# Autodesk Inventor assembly: GFRP_T2_08
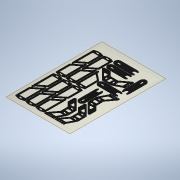
[picture p0: Inventor's stored thumbnail of the model, 180x180]
Saved by Autodesk Inventor 2020 (Build 240168000, 168)
## iProperties
Created: 2021-08-27
Part Number: GFRP_T2_08
Document SubType Name: Assembly
Designer: Masato
Author: Masato
## Documents named in this file (5)
- C:\Users\naoki\Documents\Inventor\CitBrains\git_clone\SUSTAINA_ver1_0\A_T2_175\SUSTAINA-OP\Cam\GFRP_T2_08.iam
- C:\Users\naoki\Documents\Inventor\CitBrains\git_clone\SUSTAINA_ver1_0\A_T2_175\SUSTAINA-OP\Cam\DisposableBoard.ipt
- C:\Users\naoki\Documents\Inventor\CitBrains\git_clone\SUSTAINA_ver1_0\A_T2_175\SUSTAINA-OP\UpperBody\Arm\UpperArm_side_frame.ipt
- C:\Users\naoki\Documents\Inventor\CitBrains\git_clone\SUSTAINA_ver1_0\A_T2_175\SUSTAINA-OP\UpperBody\Head\Head_side_frame.ipt
- C:\Users\naoki\Documents\Inventor\CitBrains\git_clone\SUSTAINA_ver1_0\A_T2_175\SUSTAINA-OP\UpperBody\Arm\ForeArm_inside_frame.ipt
## Components (21 placed, 4 different names)
1. DisposableBoard:1 — メイト:2, メイト:1, フラッシュ:1, フラッシュ:2, フラッシュ:3, メイト:4, メイト:5, フラッシュ:4, メイト:11, メイト:12, メイト:17, フラッシュ:7, メイト:28, メイト:29, メイト:30, フラッシュ:9, メイト:31, メイト:36, メイト:38, メイト:41, メイト:43, メイト:46
2. Head_side_frame:1 — メイト:12, フラッシュ:7, フラッシュ:8, メイト:24, メイト:34, 正接:3
3. Head_side_frame:2 — メイト:11, フラッシュ:8, メイト:24, メイト:26, フラッシュ:11
4. Head_side_frame:3 — メイト:17, メイト:26, メイト:37, フラッシュ:11, メイト:39
5. Head_side_frame:4 — メイト:29, メイト:40, 正接:5, メイト:42, メイト:45
6. UpperArm_side_frame:9 — メイト:30, フラッシュ:9, 正接:2, フラッシュ:10, メイト:34, メイト:35
7. UpperArm_side_frame:10 — 正接:2, メイト:31, フラッシュ:10, メイト:32
8. UpperArm_side_frame:11 — メイト:28, メイト:32, メイト:33, 正接:4
9. ForeArm_inside_frame:1 — メイト:36, 正接:3, メイト:37
10. ForeArm_inside_frame:2 — メイト:38, メイト:39, 正接:4, メイト:40, 正接:8
11. ForeArm_inside_frame:3 — メイト:45, メイト:46, 正接:8
12. ForeArm_inside_frame:4 — メイト:41, メイト:42, 正接:6, メイト:44
13. ForeArm_inside_frame:5 — 正接:7, メイト:43, メイト:44
14. UpperArm_side_frame:1 — メイト:5, フラッシュ:5, 正接:1
15. UpperArm_side_frame:2 — フラッシュ:3, メイト:4, フラッシュ:4, フラッシュ:5, 正接:1
16. UpperArm_side_frame:3
17. UpperArm_side_frame:4
18. UpperArm_side_frame:5
19. UpperArm_side_frame:6 — メイト:35
20. UpperArm_side_frame:7 — 正接:5, 正接:6, 正接:7
21. UpperArm_side_frame:8 — メイト:33
## Component patterns: (4 elements, first: UpperArm_side_frame:1 + UpperArm_side_frame:2)
## Relationships (46: Mate 28, Flush 10, Tangent 8)
- メイト:2 [Mate]: DisposableBoard:1
- メイト:1 [Mate]: DisposableBoard:1
- フラッシュ:1 [Flush]: DisposableBoard:1
- フラッシュ:2 [Flush]: DisposableBoard:1
- フラッシュ:3 [Flush] (2 mm): DisposableBoard:1 ↔ UpperArm_side_frame:2
- メイト:4 [Mate]: DisposableBoard:1 ↔ UpperArm_side_frame:2
- メイト:5 [Mate]: DisposableBoard:1 ↔ UpperArm_side_frame:1
- フラッシュ:4 [Flush] (2 mm): DisposableBoard:1 ↔ UpperArm_side_frame:2
- フラッシュ:5 [Flush]: UpperArm_side_frame:1 ↔ UpperArm_side_frame:2
- 正接:1 [Tangent] (2.5 mm): UpperArm_side_frame:1 ↔ UpperArm_side_frame:2
- メイト:11 [Mate]: DisposableBoard:1 ↔ Head_side_frame:2
- メイト:12 [Mate]: DisposableBoard:1 ↔ Head_side_frame:1
- メイト:17 [Mate]: DisposableBoard:1 ↔ Head_side_frame:3
- フラッシュ:7 [Flush] (2 mm): DisposableBoard:1 ↔ Head_side_frame:1
- フラッシュ:8 [Flush]: Head_side_frame:1 ↔ Head_side_frame:2
- メイト:24 [Mate] (3 mm): Head_side_frame:1 ↔ Head_side_frame:2
- メイト:26 [Mate] (2.5 mm): Head_side_frame:2 ↔ Head_side_frame:3
- メイト:28 [Mate]: DisposableBoard:1 ↔ UpperArm_side_frame:11
- メイト:29 [Mate]: DisposableBoard:1 ↔ Head_side_frame:4
- メイト:30 [Mate]: DisposableBoard:1 ↔ UpperArm_side_frame:9
- フラッシュ:9 [Flush] (2 mm): DisposableBoard:1 ↔ UpperArm_side_frame:9
- 正接:2 [Tangent] (2.5 mm): UpperArm_side_frame:9 ↔ UpperArm_side_frame:10
- メイト:31 [Mate]: DisposableBoard:1 ↔ UpperArm_side_frame:10
- フラッシュ:10 [Flush]: UpperArm_side_frame:9 ↔ UpperArm_side_frame:10
- メイト:32 [Mate] (2.5 mm): UpperArm_side_frame:10 ↔ UpperArm_side_frame:11
- メイト:33 [Mate] (2.5 mm): UpperArm_side_frame:11 ↔ UpperArm_side_frame:8
- メイト:34 [Mate] (2.5 mm): Head_side_frame:1 ↔ UpperArm_side_frame:9
- メイト:35 [Mate] (2.5 mm): UpperArm_side_frame:9 ↔ UpperArm_side_frame:6
- メイト:36 [Mate]: DisposableBoard:1 ↔ ForeArm_inside_frame:1
- 正接:3 [Tangent] (2.5 mm): Head_side_frame:1 ↔ ForeArm_inside_frame:1
- メイト:37 [Mate] (2.5 mm): Head_side_frame:3 ↔ ForeArm_inside_frame:1
- フラッシュ:11 [Flush]: Head_side_frame:2 ↔ Head_side_frame:3
- メイト:38 [Mate]: DisposableBoard:1 ↔ ForeArm_inside_frame:2
- メイト:39 [Mate] (2.5 mm): Head_side_frame:3 ↔ ForeArm_inside_frame:2
- 正接:4 [Tangent] (2.5 mm): UpperArm_side_frame:11 ↔ ForeArm_inside_frame:2
- メイト:40 [Mate] (2.5 mm): Head_side_frame:4 ↔ ForeArm_inside_frame:2
- 正接:5 [Tangent] (2.5 mm): Head_side_frame:4 ↔ UpperArm_side_frame:7
- メイト:41 [Mate]: DisposableBoard:1 ↔ ForeArm_inside_frame:4
- メイト:42 [Mate] (2.5 mm): Head_side_frame:4 ↔ ForeArm_inside_frame:4
- 正接:6 [Tangent] (2.5 mm): ForeArm_inside_frame:4 ↔ UpperArm_side_frame:7
- 正接:7 [Tangent] (2.5 mm): ForeArm_inside_frame:5 ↔ UpperArm_side_frame:7
- メイト:43 [Mate]: DisposableBoard:1 ↔ ForeArm_inside_frame:5
- メイト:44 [Mate] (2.5 mm): ForeArm_inside_frame:4 ↔ ForeArm_inside_frame:5
- メイト:45 [Mate] (2.5 mm): Head_side_frame:4 ↔ ForeArm_inside_frame:3
- メイト:46 [Mate]: DisposableBoard:1 ↔ ForeArm_inside_frame:3
- 正接:8 [Tangent] (2.5 mm): ForeArm_inside_frame:2 ↔ ForeArm_inside_frame:3
